# Autodesk Inventor assembly: SirHexAlot
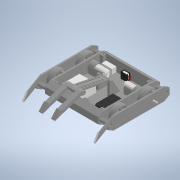
[picture p0: Inventor's stored thumbnail of the model, 180x180]
Saved by Autodesk Inventor 2020 (Build 240168000, 168)
## iProperties
Created: 2023-12-21
Part Number: SirHexAlot
Document SubType Name: Assembly
Designer: smz3rm
Mass: 440.196 g
Surface Area: 1683.01 cm^2
Volume: 343.803 cm^3
Density: 1.28037 g/cm^3
Author: smz3rm
## Documents named in this file (16)
- C:\Users\smz3rm\OneDrive - BP\Documents\DigitalTwin\Models\BattleBot\Flipper\SirHexAlot.iam
- C:\Users\smz3rm\OneDrive - BP\Documents\DigitalTwin\Models\BattleBot\Flipper\HexBody.ipt
- C:\Users\smz3rm\OneDrive - BP\Documents\DigitalTwin\Models\BattleBot\Flipper\PulleyedWheelV1.ipt
- C:\Users\smz3rm\OneDrive - BP\Documents\DigitalTwin\Models\BattleBot\DriveMotorV2.ipt
- C:\Users\smz3rm\OneDrive - BP\Documents\DigitalTwin\Models\BattleBot\SwitchHolder.ipt
- C:\Users\smz3rm\OneDrive - BP\Documents\DigitalTwin\Models\BattleBot\Switch.ipt
- C:\Users\smz3rm\OneDrive - BP\Documents\DigitalTwin\Models\BattleBot\BatteryV1.ipt
- C:\Users\smz3rm\OneDrive - BP\Documents\DigitalTwin\Models\BattleBot\Flipper\Servo.ipt
- C:\Users\smz3rm\OneDrive - BP\Documents\DigitalTwin\Models\BattleBot\Flipper\PulleyedBearingWheelV1.ipt
- C:\Users\smz3rm\OneDrive - BP\Documents\DigitalTwin\Models\BattleBot\Flipper\WheelBearings.ipt
- C:\Users\smz3rm\OneDrive - BP\Documents\DigitalTwin\Models\BattleBot\Flipper\FlipperRod.ipt
- C:\Users\smz3rm\OneDrive - BP\Documents\DigitalTwin\Models\BattleBot\Flipper\HexFlipper.ipt
- C:\Users\smz3rm\OneDrive - BP\Documents\DigitalTwin\Models\BattleBot\Flipper\HexFlipperSpike.ipt
- C:\Users\smz3rm\OneDrive - BP\Documents\DigitalTwin\Models\BattleBot\Flipper\HexWheelGuardLeft.ipt
- C:\Users\smz3rm\OneDrive - BP\Documents\DigitalTwin\Models\BattleBot\Flipper\HexWheelGuardRight.ipt
- C:\Users\smz3rm\OneDrive - BP\Documents\DigitalTwin\Models\BattleBot\FS2A.ipt
## Components (22 placed, 15 different names)
1. HexBody:1 — Mate:3, Mate:4, Mate:5, Mate:6, Mate:7, Mate:8, Mate:9, Mate:11, Mate:14, Mate:22, Mate:23, Mate:24, Mate:39, Mate:41, Mate:42, Mate:48, Mate:51, Mate:52, Mate:53, Mate:62, Flush:1, Mate:63, Mate:64, Mate:67, Mate:68, Mate:69, Mate:72, Mate:73, Mate:80, Mate:81, Mate:82
2. PulleyedWheelV1:1 — Mate:10, Mate:11
3. DriveMotorV2:1 — Mate:7, Mate:8, Mate:9, Mate:10, Mate:65
4. DriveMotorV2:2 — Mate:4, Mate:5, Mate:6, Mate:15, Mate:70
5. SwitchHolder:1 — Mate:19, Mate:20, Mate:21, Mate:22, Mate:23
6. Switch:1 — Mate:19, Mate:20, Mate:21
7. BatteryV1:1 — Mate:24, Mate:52, Mate:53
8. PulleyedWheelV1:5 — Mate:14, Mate:15
9. Servo:1 — Mate:3
10. PulleyedBearingWheelV1:1 — Mate:31, Mate:32, Mate:33, Mate:34, Mate:42
11. PulleyedBearingWheelV1:2 — Mate:35, Mate:36, Mate:37, Mate:38, Mate:39, Mate:72
12. WheelBearings:1 — Mate:31, Mate:32, Mate:66
13. WheelBearings:2 — Mate:33, Mate:34, Mate:41
14. WheelBearings:3 — Mate:35, Mate:36
15. WheelBearings:4 — Mate:37, Mate:38, Mate:71
16. FlipperRod:1 — Mate:49, Mate:50
17. HexFlipper:1 — Mate:49, Mate:50, Mate:51, Mate:62, Mate:74, Mate:75, Mate:76, Mate:77, Mate:78, Mate:79
18. HexFlipperSpike:1 — Mate:77, Mate:78, Mate:79
19. HexFlipperSpike:2 — Mate:74, Mate:75, Mate:76
20. HexWheelGuardLeft:1 — Mate:63, Mate:64, Mate:65, Mate:66, Mate:67
21. HexWheelGuardRight:1 — Mate:68, Mate:69, Mate:70, Mate:71, Mate:73
22. FS2A:1 — Mate:80, Mate:81, Mate:82
## Relationships (56: Mate 55, Flush 1)
- Mate:3: HexBody:1 ↔ Servo:1
- Mate:4: HexBody:1 ↔ DriveMotorV2:2
- Mate:5: HexBody:1 ↔ DriveMotorV2:2
- Mate:6: HexBody:1 ↔ DriveMotorV2:2
- Mate:7: HexBody:1 ↔ DriveMotorV2:1
- Mate:8: HexBody:1 ↔ DriveMotorV2:1
- Mate:9: HexBody:1 ↔ DriveMotorV2:1
- Mate:10: PulleyedWheelV1:1 ↔ DriveMotorV2:1
- Mate:11: HexBody:1 ↔ PulleyedWheelV1:1
- Mate:14: HexBody:1 ↔ PulleyedWheelV1:5
- Mate:15: DriveMotorV2:2 ↔ PulleyedWheelV1:5
- Mate:19: SwitchHolder:1 ↔ Switch:1
- Mate:20: SwitchHolder:1 ↔ Switch:1
- Mate:21: SwitchHolder:1 ↔ Switch:1
- Mate:22: HexBody:1 ↔ SwitchHolder:1
- Mate:23: HexBody:1 ↔ SwitchHolder:1
- Mate:24: HexBody:1 ↔ BatteryV1:1
- Mate:31: PulleyedBearingWheelV1:1 ↔ WheelBearings:1
- Mate:32: PulleyedBearingWheelV1:1 ↔ WheelBearings:1
- Mate:33: PulleyedBearingWheelV1:1 ↔ WheelBearings:2
- Mate:34: PulleyedBearingWheelV1:1 ↔ WheelBearings:2
- Mate:35: PulleyedBearingWheelV1:2 ↔ WheelBearings:3
- Mate:36: PulleyedBearingWheelV1:2 ↔ WheelBearings:3
- Mate:37: PulleyedBearingWheelV1:2 ↔ WheelBearings:4
- Mate:38: PulleyedBearingWheelV1:2 ↔ WheelBearings:4
- Mate:39: HexBody:1 ↔ PulleyedBearingWheelV1:2
- Mate:41: HexBody:1 ↔ WheelBearings:2
- Mate:42: HexBody:1 ↔ PulleyedBearingWheelV1:1
- Mate:48: HexBody:1
- Mate:49: FlipperRod:1 ↔ HexFlipper:1
- Mate:50: FlipperRod:1 ↔ HexFlipper:1
- Mate:51: HexBody:1 ↔ HexFlipper:1
- Mate:52: HexBody:1 ↔ BatteryV1:1
- Mate:53: HexBody:1 ↔ BatteryV1:1
- Mate:62 (1 mm): HexBody:1 ↔ HexFlipper:1
- Flush:1: HexBody:1
- Mate:63: HexBody:1 ↔ HexWheelGuardLeft:1
- Mate:64: HexBody:1 ↔ HexWheelGuardLeft:1
- Mate:65: DriveMotorV2:1 ↔ HexWheelGuardLeft:1
- Mate:66: WheelBearings:1 ↔ HexWheelGuardLeft:1
- Mate:67: HexBody:1 ↔ HexWheelGuardLeft:1
- Mate:68: HexBody:1 ↔ HexWheelGuardRight:1
- Mate:69: HexBody:1 ↔ HexWheelGuardRight:1
- Mate:70: DriveMotorV2:2 ↔ HexWheelGuardRight:1
- Mate:71: WheelBearings:4 ↔ HexWheelGuardRight:1
- Mate:72: HexBody:1 ↔ PulleyedBearingWheelV1:2
- Mate:73: HexBody:1 ↔ HexWheelGuardRight:1
- Mate:74: HexFlipper:1 ↔ HexFlipperSpike:2
- Mate:75: HexFlipper:1 ↔ HexFlipperSpike:2
- Mate:76: HexFlipper:1 ↔ HexFlipperSpike:2
- Mate:77: HexFlipper:1 ↔ HexFlipperSpike:1
- Mate:78: HexFlipper:1 ↔ HexFlipperSpike:1
- Mate:79: HexFlipper:1 ↔ HexFlipperSpike:1
- Mate:80: HexBody:1 ↔ FS2A:1
- Mate:81: HexBody:1 ↔ FS2A:1
- Mate:82: HexBody:1 ↔ FS2A:1
